# Autodesk Inventor assembly: belt_reducer_1
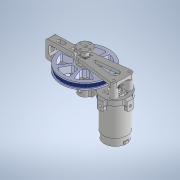
[picture p0: Inventor's stored thumbnail of the model, 180x180]
Saved by Autodesk Inventor 2020 (Build 240168000, 168)
## iProperties
Created: 2019-10-15
Part Number: belt_reducer_1
Document SubType Name: Assembly
Designer: psrob
Author: psrob
## Documents named in this file (10)
- E:\projects-2\haptic device gen3\hardware\belt_reducer_2.iam
- E:\projects-2\haptic device gen3\hardware\gt2-pulley-120-tooth-1.snapshot.1\120teeth gt2 pulley.ipt
- E:\projects-2\haptic device gen3\hardware\flange_6mm.ipt
- E:\projects-2\haptic device gen3\hardware\pin_6_60.ipt
- E:\projects-2\haptic device gen3\hardware\bearing_6_13_5.ipt
- E:\projects-2\haptic device gen3\hardware\motor_1.ipt
- E:\projects-2\haptic device gen3\hardware\GT2_16T.ipt
- E:\projects-2\haptic device gen3\hardware\motor_holder_1.ipt
- E:\projects-2\haptic device gen3\hardware\sensor_holder_1.ipt
- E:\projects-2\haptic device gen3\hardware\frame-1.ipt
## Components (11 placed, 9 different names)
1. 120teeth gt2 pulley:1 — Insert:1, Insert:2, Insert:4
2. flange_6mm:1 — Insert:1, Insert:2, Insert:3
3. pin_6_60:1 — Insert:3
4. bearing_6_13_5:1 — Insert:4, Insert:8
5. motor_1:1 — Insert:5, Flush:1, Insert:6, Insert:7
6. GT2_16T:1 — Insert:5
7. motor_holder_1:1 — Flush:1, Insert:6, Insert:7, Insert:8, Flush:2, Insert:12, Insert:13, Insert:14
8. sensor_holder_1:1 — Flush:2, Insert:11, Insert:12, Insert:13, Insert:15
9. frame-1:1 — Insert:11, Insert:14
10. bearing_6_13_5:3 — Insert:15, Insert:16
11. flange_6mm:2 — Insert:16
## Relationships (16: Insert 14, Flush 2)
- Insert:1: 120teeth gt2 pulley:1 ↔ flange_6mm:1
- Insert:2: 120teeth gt2 pulley:1 ↔ flange_6mm:1
- Insert:3 (-20 mm): flange_6mm:1 ↔ pin_6_60:1
- Insert:4: 120teeth gt2 pulley:1 ↔ bearing_6_13_5:1
- Insert:5: motor_1:1 ↔ GT2_16T:1
- Flush:1: motor_1:1 ↔ motor_holder_1:1
- Insert:6: motor_1:1 ↔ motor_holder_1:1
- Insert:7: motor_1:1 ↔ motor_holder_1:1
- Insert:8: bearing_6_13_5:1 ↔ motor_holder_1:1
- Flush:2: motor_holder_1:1 ↔ sensor_holder_1:1
- Insert:11 (0.5 mm): sensor_holder_1:1 ↔ frame-1:1
- Insert:12: motor_holder_1:1 ↔ sensor_holder_1:1
- Insert:13: motor_holder_1:1 ↔ sensor_holder_1:1
- Insert:14 (0.5 mm): motor_holder_1:1 ↔ frame-1:1
- Insert:15: sensor_holder_1:1 ↔ bearing_6_13_5:3
- Insert:16 (1 mm): bearing_6_13_5:3 ↔ flange_6mm:2
